# Autodesk Inventor assembly: Demonstrator
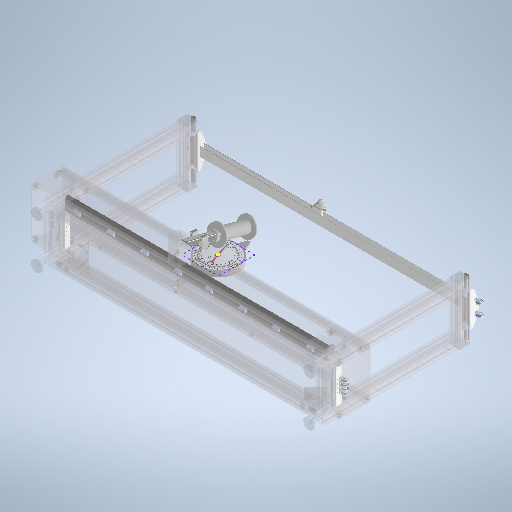
[picture p0: Inventor's stored thumbnail of the model, 512x512]
Saved by Autodesk Inventor 2025 (Build 290162010, 162A)
## iProperties
Created: 2024-11-07
Part Number: Demonstrator
Document SubType Name: Assembly
Designer: Admin
Mass: 7442.58 g
Surface Area: 46120.1 cm^2
Volume: 6360.4 cm^3
Density: 1.17015 g/cm^3
dummerWinkel: 1.5
Author: Admin
## Documents named in this file (38)
- C:\Users\Admin\GIT\HDVKBM\CAD\Krandemonstrator\Demonstrator.iam
- C:\Users\Admin\GIT\HDVKBM\CAD\Krandemonstrator\Träger.ipt
- C:\Users\Admin\Documents\Inventor\Content Center Files\R2025\de-DE\AS 1112 (2)\AS 1112 - M4  Typ 5.ipt
- C:\Users\Admin\GIT\HDVKBM\CAD\Krandemonstrator\MontageAufnahmeLO.ipt
- C:\Users\Admin\Documents\Inventor\Content Center Files\R2025\de-DE\AS 1427(03)\AS 1427 - M2 x 6(1).ipt
- C:\Users\Admin\GIT\HDVKBM\CAD\Krandemonstrator\Katze.iam
- C:\Users\Admin\GIT\HDVKBM\CAD\Krandemonstrator\UmlenkrolleHalterEinfach.iam
- C:\Users\Admin\GIT\HDVKBM\CAD\Krandemonstrator\SeilStange1m.ipt
- C:\Users\Admin\GIT\HDVKBM\CAD\Krandemonstrator\RollenhalterU.ipt
- C:\Users\Admin\GIT\HDVKBM\CAD\Krandemonstrator\UmlenkrolleHalterDoppelt.iam
- C:\Users\Admin\GIT\HDVKBM\CAD\Krandemonstrator\SeilatrappeHalter.ipt
- C:\Users\Admin\GIT\HDVKBM\CAD\Krandemonstrator\UmlenkrolleHalterDoppeltAngle.iam
- C:\Users\Admin\GIT\HDVKBM\CAD\Krandemonstrator\UmlenkrolleHalterEinfachAngle.iam
- C:\Users\Admin\GIT\HDVKBM\CAD\Krandemonstrator\UmlenkrolleHalterEinfachAngleB.iam
- C:\Users\Admin\GIT\HDVKBM\CAD\Krandemonstrator\seilatrappeHalterMini.ipt
- C:\Users\Admin\Documents\Inventor\Content Center Files\R2025\de-DE\AS 1421(4)\AS 1421 - M4 x 8 Kegelstumpf.ipt
- C:\Users\Admin\GIT\HDVKBM\CAD\Krandemonstrator\WS_10_40_930_2\WS_10_40_930_2.iam
- C:\Users\Admin\GIT\HDVKBM\CAD\Krandemonstrator\Frame.iam
- C:\Users\Admin\GIT\HDVKBM\CAD\Krandemonstrator\item_42006_nutenstein-8-st-m4-verzi__high\item_42006_nutenstein-8-st-m4-verzi__high.ipt
- C:\Users\Admin\Documents\Inventor\Content Center Files\R2025\de-DE\DIN 7991(2)\DIN 7991 - M4x30.ipt
- C:\Users\Admin\GIT\HDVKBM\CAD\Krandemonstrator\item_2623_nutenstein-8-st-m6-verzi__high\item_2623_nutenstein-8-st-m6-verzi__high.ipt
- C:\Users\Admin\Documents\Inventor\Content Center Files\R2025\de-DE\DIN 7991(2)\DIN 7991 - M6x16.ipt
- C:\Users\Admin\GIT\HDVKBM\CAD\Krandemonstrator\Zugfeder11.ipt
- C:\Users\Admin\GIT\HDVKBM\CAD\Krandemonstrator\Bedienhebel.iam
- C:\Users\Admin\Documents\Inventor\Content Center Files\R2025\de-DE\DIN 7991(1)\DIN 7991 - M4  x  25.ipt
- C:\Users\Admin\Documents\Inventor\Content Center Files\R2025\de-DE\DIN 7991(2)\DIN 7991 - M4x25.ipt
- C:\Users\Admin\GIT\HDVKBM\CAD\Krandemonstrator\SeilStange3cm.ipt
- C:\Users\Admin\GIT\HDVKBM\CAD\Krandemonstrator\waage.ipt
- C:\Users\Admin\GIT\HDVKBM\CAD\Krandemonstrator\verkleidungBremse.ipt
- C:\Users\Admin\Documents\Inventor\Content Center Files\R2025\de-DE\AS 1427(03)\AS 1427 - M2 x 4(1).ipt
- C:\Users\Admin\GIT\HDVKBM\CAD\Krandemonstrator\Platte Scharfe Ecken (mm) 150 x 30 x 8.ipt
- C:\Users\Admin\Documents\Inventor\Content Center Files\R2025\de-DE\DIN EN ISO 7089\DIN EN ISO 7089 -  5.ipt
- C:\Users\Admin\Documents\Inventor\Content Center Files\R2025\de-DE\DIN 933\DIN 933 - M5  x 8.ipt
- C:\Users\Admin\GIT\HDVKBM\CAD\Krandemonstrator\item_42005_nutenstein-8-st-m5-verzi__high\item_42005_nutenstein-8-st-m5-verzi__high.ipt
- C:\Users\Admin\Documents\Inventor\Content Center Files\R2025\de-DE\DIN 933\DIN 933 - M5  x 18.ipt
- C:\Users\Admin\GIT\HDVKBM\CAD\Krandemonstrator\MontageAufnahmeLO-LH.ipt
- C:\Users\Admin\Documents\Inventor\Content Center Files\R2025\de-DE\DIN 7991(1)\DIN 7991 - M3  x  16.ipt
- C:\Users\Admin\Documents\Inventor\Content Center Files\R2025\de-DE\DIN 7991(1)\DIN 7991 - M3  x  25.ipt
## Components (138 placed, 40 different names)
1. Katze:1 [sub-assembly] — KatzeLagerHO, KatzeLagerVV, KatzeSeilMutterVL, KatzeSeilMutterHL, KatzeSeilMutterVR, KatzeSeilMutterHR, KatzeGewindeSeilStumpfVL, KatzeGewindeSeilStumpfHL, KatzeGewindeSeilStumpfVR, KatzeGewindeSeilStumpfHR, KatzeSeilStumpfVL, KatzeSeilStumpfHL, KatzeSeilStumpfVR, KatzeSeilStumpfHR, Zylindrisch:83
2. Frame:1 [sub-assembly] — Starr:83, Starr:88, Starr:89, Starr:124, Starr:134, Starr:136
3. DIN EN ISO 7089 5:1
4. DIN EN ISO 7089 5:2
5. DIN EN ISO 7089 5:3
6. DIN EN ISO 7089 5:4
7. DIN 933 - ersetzt durch DIN EN 24017 M5  x 8:1
8. DIN 933 - ersetzt durch DIN EN 24017 M5  x 8:2 — Zylindrisch:109
9. DIN 933 - ersetzt durch DIN EN 24017 M5  x 8:3
10. DIN 933 - ersetzt durch DIN EN 24017 M5  x 8:4 — Zylindrisch:110
11. Platte Scharfe Ecken (mm) 150 x 30 x 8:2 — Starr:136, Einfügen:8, Zylindrisch:110
12. Platte Scharfe Ecken (mm) 150 x 30 x 8:1 — Starr:134, Zylindrisch:109, Planar:57
13. DIN 933 - ersetzt durch DIN EN 24017 M5  x 18:2
14. DIN 933 - ersetzt durch DIN EN 24017 M5  x 18:3
15. DIN 933 - ersetzt durch DIN EN 24017 M5  x 18:4
16. DIN 933 - ersetzt durch DIN EN 24017 M5  x 18:1 — Einfügen:8
17. DIN 7991 - ersetzt durch DIN EN ISO 10642 M3  x  16:4 — Passend:17
18. DIN 7991 - ersetzt durch DIN EN ISO 10642 M3  x  25:4 — Passend:18
19. DIN 7991 - ersetzt durch DIN EN ISO 10642 M3  x  25:3 — Passend:19
20. DIN 7991 - ersetzt durch DIN EN ISO 10642 M3  x  16:3 — Passend:20
21. DIN 7991 - ersetzt durch DIN EN ISO 10642 M3  x  16:2 — Passend:21
22. DIN 7991 - ersetzt durch DIN EN ISO 10642 M3  x  25:2 — Passend:22
23. DIN 7991 - ersetzt durch DIN EN ISO 10642 M3  x  16:1 — Passend:23
24. DIN 7991 - ersetzt durch DIN EN ISO 10642 M3  x  25:1 — Passend:24
25. MontageAufnahmeLO-LH:2 — SeilrolleORHscrewA, SeilrolleORHscrewB, SeilrolleORHplan, Starr:137, Passend:21, Passend:22
26. MontageAufnahmeLO:2 — SeilrolleORVplan, SeilrolleORVscrewA, SeilrolleORVscrewB, Starr:138, Passend:23, Passend:24
27. MontageAufnahmeLOV:1 — SeilrolleOLVAuflage, SeilrolleOLVSchraubeA, SeilrolleOLVSchraubeB, Starr:140, Passend:19, Passend:20
28. MontageAufnahmeLOH:1 — SeilrolleOLHAuflage, SeilrolleOLHSchraubeA, SeilrolleOLHSchraubeB, Starr:139, Passend:17, Passend:18
29. item_42005_nutenstein-8-st-m5-verzi__high:1
30. item_42005_nutenstein-8-st-m5-verzi__high:2
31. item_42005_nutenstein-8-st-m5-verzi__high:4
32. item_42005_nutenstein-8-st-m5-verzi__high:3
33. Träger:1 — KatzeLagerHO, KatzeLagerVV, Starr:137, Starr:138, Starr:139, Starr:140, Planar:57
34. Bedienhebel:1 [sub-assembly] — Passend:5, Passend:6, Passend:7, Passend:8, Kugelförmig:1, Kugelförmig:3
35. DIN 7991 - ersetzt durch DIN EN ISO 10642 M4  x  25:1 — Passend:5
36. DIN 7991 M4x25:1 — Passend:6
37. DIN 7991 M4x25:2 — Passend:7
38. DIN 7991 M4x25:3 — Passend:8
39. verkleidungBremse:1 — Passend:15, Passend:16
40. AS 1427 - Metrisch M2 x 4:1 — Passend:15
41. AS 1427 - Metrisch M2 x 4:2 — Passend:16
42. AS 1427 - Metrisch M2 x 4:3
43. AS 1427 - Metrisch M2 x 4:4
44. DIN 7991 M6x16:1 — Starr:90, Starr:105
45. DIN 7991 M6x16:2 — Starr:91, Starr:104
46. DIN 7991 M6x16:3 — Starr:93, Starr:102
47. DIN 7991 M6x16:4 — Starr:92, Starr:103
48. DIN 7991 M6x16:5 — Starr:97, Starr:98
49. DIN 7991 M6x16:6 — Starr:96, Starr:99
50. DIN 7991 M6x16:7 — Starr:95, Starr:100
51. DIN 7991 M6x16:8 — Starr:94, Starr:101
52. item_2623_nutenstein-8-st-m6-verzi__high:1 — Starr:105
53. item_2623_nutenstein-8-st-m6-verzi__high:2 — Starr:104
54. item_2623_nutenstein-8-st-m6-verzi__high:3 — Starr:99
55. item_2623_nutenstein-8-st-m6-verzi__high:4 — Starr:103
56. item_2623_nutenstein-8-st-m6-verzi__high:5 — Starr:102
57. item_2623_nutenstein-8-st-m6-verzi__high:6 — Starr:101
58. item_2623_nutenstein-8-st-m6-verzi__high:7 — Starr:100
59. item_2623_nutenstein-8-st-m6-verzi__high:8 — Starr:98
60. WS_10_40_930_2:1 [sub-assembly] — Starr:89, Starr:90, Starr:91, Starr:92, Starr:93, Starr:94, Starr:95, Starr:96, Starr:97
61. lastseil — Zylindrisch:83, Starr:117
62. Zugfeder1:1 — Starr:118
63. waage:1 — Starr:117, Starr:118
64. SeilStange3cm:5 — Starr:119, Kugelförmig:3
65. SeilStange3cm:6 — Starr:119
66. SeilStange3cm:7 — Starr:122
67. SeilStange3cm:8 — Starr:122, Starr:123
68. SeilStange3cm:2 — Zylindrisch:108
69. SeilStange3cm:1 — Kugelförmig:1, Zylindrisch:108, Starr:123
70. seilatrappeHalterMini:3 — SeilAtrappeHalterMini3, SeilAtrappeHalterMini3Seil
71. seilatrappeHalterMini:4 — SeilAtrappeHalterMini4, SeilAtrappeHalterMini4Seil
72. SeilStange1m:16 — SeilrolleULMVsld, SeilAtrappeHalterMini3Seil
73. SeilStange1m:17 — SeilrolleULMHsld, SeilAtrappeHalterMini4Seil
74. SeilStange1m:18 — SeilAtrappeHalterMini1Seil, SeilrolleORVver, SeilrolleURMVver
75. SeilStange1m:19 — SeilAtrappeHalterMini2Seil, SeilrolleORHver, SeilrolleURMHver
76. seilatrappeHalterMini:1 — SeilAtrappeHalterMini1, SeilAtrappeHalterMini1Seil
77. seilatrappeHalterMini:2 — SeilAtrappeHalterMini2, SeilAtrappeHalterMini2Seil
78. SeilStange1m:13 — SeilrolleURHsld
79. SeilStange1m:12 — SeilrolleURVsld
80. SeilatrappeHalter:1 — SeilAtrappeHalterSeilA, SeilAtrappeHalterSeilB, Starr:124
81. SeilStange1m:1 — KatzeGewindeSeilStumpfVL, SeilrolleOLVhor
82. SeilStange1m:3 — SeilrolleOLHhor, KatzeSeilStumpfHL
83. SeilStange1m:4 — SeilrolleORHhor, KatzeSeilStumpfHR
84. SeilStange1m:5 — SeilrolleORVhor, KatzeSeilStumpfVR
85. SeilStange1m:8 — SeilAtrappeHalterSeilB, SeilrolleOLHver, SeilrolleULHver
86. SeilStange1m:9 — SeilAtrappeHalterSeilA, SeilrolleOLVver, SeilrolleULVver
87. SeilStange1m:10 — Zylindrisch:15, SeilrolleULHhor, SeilrolleURHhor
88. SeilStange1m:11 — Zylindrisch:16, SeilrolleULVhor, SeilrolleURVhor
89. SeilStange1m:14 — SeilAtrappeRollenhalterSeilB, SeilrolleULMHhor, SeilrolleURMHhor
90. SeilStange1m:15 — SeilAtrappeRollenhalterSeilA, SeilrolleULMVhor, SeilrolleURMVhor
91. AS 1427 - Metrisch M2 x 6:2 — SeilrolleOLVSchraube2, SeilrolleOLVSchraubeA
92. AS 1427 - Metrisch M2 x 6:1 — SeilrolleOLVSchraube1, SeilrolleOLVSchraubeB
93. UmlenkrolleHalterEinfach:1 [sub-assembly] — SeilrolleOLVSchraube1, SeilrolleOLVAuflage, SeilrolleOLVSchraube2, SeilrolleOLVhor, SeilrolleOLVver
94. AS 1427 - Metrisch M2 x 6:3 — SeilrolleOLHSchraube1, SeilrolleOLHSchraubeA
95. AS 1427 - Metrisch M2 x 6:4 — SeilrolleOLHSchraube2, SeilrolleOLHSchraubeB
96. UmlenkrolleHalterEinfach:2 [sub-assembly] — SeilrolleOLHSchraube1, SeilrolleOLHSchraube2, SeilrolleOLHAuflage, SeilrolleOLHhor, SeilrolleOLHver
97. AS 1112 (2) - Metrisch M4  Typ 5:4 — KatzeSeilMutterVR
98. AS 1112 (2) - Metrisch M4  Typ 5:3 — KatzeSeilMutterVL
99. AS 1112 (2) - Metrisch M4  Typ 5:2 — KatzeSeilMutterHR
100. AS 1112 (2) - Metrisch M4  Typ 5:1 — KatzeSeilMutterHL
101. AS 1421 Kegelstumpf - Metrisch M4 x 8 Kegelstumpf:4 — KatzeGewindeSeilStumpfHR
102. AS 1421 Kegelstumpf - Metrisch M4 x 8 Kegelstumpf:1 — KatzeGewindeSeilStumpfVR
103. AS 1421 Kegelstumpf - Metrisch M4 x 8 Kegelstumpf:2 — KatzeSeilStumpfVL
104. AS 1421 Kegelstumpf - Metrisch M4 x 8 Kegelstumpf:3 — KatzeGewindeSeilStumpfHL
105. UmlenkrolleHalterEinfachAngle:1 [sub-assembly] — SeilrolleORVscrewAfix, SeilrolleORVscrewBfix, SeilrolleORVplan, SeilrolleORVhor, SeilrolleORVver, SeilAtrappeHalterMini1
106. AS 1427 - Metrisch M2 x 6:17 — SeilrolleORVscrewBfix, SeilrolleORVscrewB
107. AS 1427 - Metrisch M2 x 6:18 — SeilrolleORVscrewAfix, SeilrolleORVscrewA
108. AS 1427 - Metrisch M2 x 6:19 — SeilrolleORHscrewB, SeilrolleORHscrewBfix
109. AS 1427 - Metrisch M2 x 6:20 — SeilrolleORHscrewA, SeilrolleORHscrewAfix
110. UmlenkrolleHalterEinfachAngleB:1 [sub-assembly] — SeilrolleORHplan, SeilrolleORHscrewAfix, SeilrolleORHscrewBfix, SeilAtrappeHalterMini2, SeilrolleORHhor, SeilrolleORHver
111. RollenhalterU:1 — Planar:24, Zylindrisch:5, Zylindrisch:6, Planar:25, Zylindrisch:7, Zylindrisch:8, Planar:40, Zylindrisch:9, Zylindrisch:10, Zylindrisch:15, Zylindrisch:16, Starr:84, Starr:85, Passend:1, Passend:2, Starr:88
112. DIN 7991 M4x30:1 — Passend:1
113. DIN 7991 M4x30:2 — Passend:2
114. UmlenkrolleHalterDoppelt:1 [sub-assembly] — Planar:24, Starr:33, Starr:34, SeilrolleULMHhor, SeilrolleULMVhor, SeilrolleULMHsld, SeilrolleULMVsld, SeilAtrappeHalterMini3, SeilAtrappeHalterMini4
115. UmlenkrolleHalterEinfach:3 [sub-assembly] — Starr:35, Starr:36, Planar:25, SeilrolleULVver, SeilrolleULVhor
116. UmlenkrolleHalterEinfach:4 [sub-assembly] — Starr:37, Starr:38, Planar:40, SeilrolleULHver, SeilrolleULHhor
117. AS 1427 - Metrisch M2 x 6:5 — Starr:38, Zylindrisch:9
118. AS 1427 - Metrisch M2 x 6:6 — Starr:37, Zylindrisch:10
119. AS 1427 - Metrisch M2 x 6:7 — Starr:34, Zylindrisch:6
120. AS 1427 - Metrisch M2 x 6:8 — Starr:33, Zylindrisch:5
121. AS 1427 - Metrisch M2 x 6:9 — Starr:35, Zylindrisch:8
122. item_42006_nutenstein-8-st-m4-verzi__high:1 — Starr:85
123. item_42006_nutenstein-8-st-m4-verzi__high:2 — Starr:84
124. AS 1427 - Metrisch M2 x 6:10 — Starr:36, Zylindrisch:7
125. UmlenkrolleHalterEinfach:5 [sub-assembly] — Starr:45, Starr:44, Planar:42, SeilrolleURVhor, SeilrolleURVsld
126. UmlenkrolleHalterEinfach:6 [sub-assembly] — Starr:46, Starr:47, Planar:43, SeilrolleURHhor, SeilrolleURHsld
127. UmlenkrolleHalterDoppeltAngle:1 [sub-assembly] — Planar:54, Starr:53, Starr:54, SeilrolleURMHhor, SeilrolleURMVhor, SeilrolleURMVver, SeilrolleURMHver
128. AS 1427 - Metrisch M2 x 6:11 — Starr:47, Zylindrisch:22
129. AS 1427 - Metrisch M2 x 6:12 — Starr:46, Zylindrisch:21
130. AS 1427 - Metrisch M2 x 6:13 — Starr:45, Zylindrisch:20
131. AS 1427 - Metrisch M2 x 6:14 — Zylindrisch:18, Starr:53
132. AS 1427 - Metrisch M2 x 6:15 — Zylindrisch:17, Starr:54
133. AS 1427 - Metrisch M2 x 6:16 — Starr:44, Zylindrisch:19
134. RollenhalterU:2 — Zylindrisch:17, Zylindrisch:18, Planar:42, Zylindrisch:19, Zylindrisch:20, Planar:43, Zylindrisch:21, Zylindrisch:22, Planar:54, SeilAtrappeRollenhalterSeilB, SeilAtrappeRollenhalterSeilA, Starr:83, Passend:3, Passend:4, Starr:86, Starr:87
135. DIN 7991 M4x30:3 — Passend:3
136. item_42006_nutenstein-8-st-m4-verzi__high:3 — Starr:87
137. item_42006_nutenstein-8-st-m4-verzi__high:4 — Starr:86
138. DIN 7991 M4x30:4 — Passend:4
## Relationships (174: WeldJoint 75, CylindricalJoint 34, RelateRotateTranslate 24, Mate 18, PlanarJoint 13, Insert 8, BallJoint 2)
- KatzeLagerHO [PlanarJoint] (0.05 mm): Katze:1 ↔ Träger:1
- KatzeLagerVV [PlanarJoint] (0.05 mm): Katze:1 ↔ Träger:1
- KatzeSeilMutterVL [WeldJoint]: Katze:1 ↔ AS 1112 (2) - Metrisch M4  Typ 5:3
- KatzeSeilMutterHL [WeldJoint]: Katze:1 ↔ AS 1112 (2) - Metrisch M4  Typ 5:1
- KatzeSeilMutterVR [WeldJoint]: Katze:1 ↔ AS 1112 (2) - Metrisch M4  Typ 5:4
- KatzeSeilMutterHR [WeldJoint]: Katze:1 ↔ AS 1112 (2) - Metrisch M4  Typ 5:2
- KatzeGewindeSeilStumpfVL [WeldJoint]: Katze:1 ↔ SeilStange1m:1
- KatzeGewindeSeilStumpfHL [WeldJoint]: Katze:1 ↔ AS 1421 Kegelstumpf - Metrisch M4 x 8 Kegelstumpf:3
- KatzeGewindeSeilStumpfVR [WeldJoint]: Katze:1 ↔ AS 1421 Kegelstumpf - Metrisch M4 x 8 Kegelstumpf:1
- KatzeGewindeSeilStumpfHR [WeldJoint]: Katze:1 ↔ AS 1421 Kegelstumpf - Metrisch M4 x 8 Kegelstumpf:4
- KatzeSeilStumpfVL [WeldJoint]: Katze:1 ↔ AS 1421 Kegelstumpf - Metrisch M4 x 8 Kegelstumpf:2
- KatzeSeilStumpfHL [WeldJoint]: Katze:1 ↔ SeilStange1m:3
- KatzeSeilStumpfVR [WeldJoint]: Katze:1 ↔ SeilStange1m:5
- KatzeSeilStumpfHR [WeldJoint]: Katze:1 ↔ SeilStange1m:4
- SeilrolleOLVSchraube1 [WeldJoint]: AS 1427 - Metrisch M2 x 6:1 ↔ UmlenkrolleHalterEinfach:1
- SeilrolleOLVSchraube2 [WeldJoint]: AS 1427 - Metrisch M2 x 6:2 ↔ UmlenkrolleHalterEinfach:1
- SeilrolleOLVAuflage [PlanarJoint]: MontageAufnahmeLOV:1 ↔ UmlenkrolleHalterEinfach:1
- SeilrolleOLVSchraubeA [CylindricalJoint]: MontageAufnahmeLOV:1 ↔ AS 1427 - Metrisch M2 x 6:2
- SeilrolleOLVSchraubeB [CylindricalJoint]: MontageAufnahmeLOV:1 ↔ AS 1427 - Metrisch M2 x 6:1
- SeilrolleOLVhor [RelateRotateTranslate] (9 mm): SeilStange1m:1 ↔ UmlenkrolleHalterEinfach:1
- SeilrolleOLVver [RelateRotateTranslate] (9 mm): SeilStange1m:9 ↔ UmlenkrolleHalterEinfach:1
- SeilrolleOLHSchraube1 [WeldJoint]: AS 1427 - Metrisch M2 x 6:3 ↔ UmlenkrolleHalterEinfach:2
- SeilrolleOLHSchraube2 [WeldJoint]: AS 1427 - Metrisch M2 x 6:4 ↔ UmlenkrolleHalterEinfach:2
- SeilrolleOLHAuflage [PlanarJoint]: MontageAufnahmeLOH:1 ↔ UmlenkrolleHalterEinfach:2
- SeilrolleOLHSchraubeA [CylindricalJoint]: MontageAufnahmeLOH:1 ↔ AS 1427 - Metrisch M2 x 6:3
- SeilrolleOLHSchraubeB [CylindricalJoint]: MontageAufnahmeLOH:1 ↔ AS 1427 - Metrisch M2 x 6:4
- SeilrolleOLHhor [RelateRotateTranslate] (9 mm): SeilStange1m:3 ↔ UmlenkrolleHalterEinfach:2
- SeilrolleOLHver [RelateRotateTranslate] (9 mm): SeilStange1m:8 ↔ UmlenkrolleHalterEinfach:2
- Planar:24: RollenhalterU:1 ↔ UmlenkrolleHalterDoppelt:1
- Starr:33 [WeldJoint]: UmlenkrolleHalterDoppelt:1 ↔ AS 1427 - Metrisch M2 x 6:8
- Starr:34 [WeldJoint]: UmlenkrolleHalterDoppelt:1 ↔ AS 1427 - Metrisch M2 x 6:7
- Zylindrisch:5 [CylindricalJoint]: RollenhalterU:1 ↔ AS 1427 - Metrisch M2 x 6:8
- Zylindrisch:6 [CylindricalJoint]: RollenhalterU:1 ↔ AS 1427 - Metrisch M2 x 6:7
- Starr:35 [WeldJoint]: UmlenkrolleHalterEinfach:3 ↔ AS 1427 - Metrisch M2 x 6:9
- Starr:36 [WeldJoint]: UmlenkrolleHalterEinfach:3 ↔ AS 1427 - Metrisch M2 x 6:10
- Planar:25: RollenhalterU:1 ↔ UmlenkrolleHalterEinfach:3
- Zylindrisch:7 [CylindricalJoint]: RollenhalterU:1 ↔ AS 1427 - Metrisch M2 x 6:10
- Zylindrisch:8 [CylindricalJoint]: RollenhalterU:1 ↔ AS 1427 - Metrisch M2 x 6:9
- Starr:37 [WeldJoint]: UmlenkrolleHalterEinfach:4 ↔ AS 1427 - Metrisch M2 x 6:6
- Starr:38 [WeldJoint]: UmlenkrolleHalterEinfach:4 ↔ AS 1427 - Metrisch M2 x 6:5
- Planar:40: RollenhalterU:1 ↔ UmlenkrolleHalterEinfach:4
- Zylindrisch:9 [CylindricalJoint]: RollenhalterU:1 ↔ AS 1427 - Metrisch M2 x 6:5
- Zylindrisch:10 [CylindricalJoint]: RollenhalterU:1 ↔ AS 1427 - Metrisch M2 x 6:6
- SeilAtrappeHalterSeilA [CylindricalJoint]: SeilatrappeHalter:1 ↔ SeilStange1m:9
- SeilAtrappeHalterSeilB [CylindricalJoint]: SeilatrappeHalter:1 ↔ SeilStange1m:8
- Zylindrisch:15 [CylindricalJoint]: SeilStange1m:10 ↔ RollenhalterU:1
- Zylindrisch:16 [CylindricalJoint]: SeilStange1m:11 ↔ RollenhalterU:1
- SeilrolleULVver [RelateRotateTranslate] (9 mm): SeilStange1m:9 ↔ UmlenkrolleHalterEinfach:3
- SeilrolleULHver [RelateRotateTranslate] (9 mm): SeilStange1m:8 ↔ UmlenkrolleHalterEinfach:4
- SeilrolleULVhor [RelateRotateTranslate] (9 mm): SeilStange1m:11 ↔ UmlenkrolleHalterEinfach:3
- SeilrolleULHhor [RelateRotateTranslate] (9 mm): SeilStange1m:10 ↔ UmlenkrolleHalterEinfach:4
- Zylindrisch:17 [CylindricalJoint]: AS 1427 - Metrisch M2 x 6:15 ↔ RollenhalterU:2
- Zylindrisch:18 [CylindricalJoint]: AS 1427 - Metrisch M2 x 6:14 ↔ RollenhalterU:2
- Starr:45 [WeldJoint]: UmlenkrolleHalterEinfach:5 ↔ AS 1427 - Metrisch M2 x 6:13
- Starr:44 [WeldJoint]: UmlenkrolleHalterEinfach:5 ↔ AS 1427 - Metrisch M2 x 6:16
- Planar:42: UmlenkrolleHalterEinfach:5 ↔ RollenhalterU:2
- Zylindrisch:19 [CylindricalJoint]: AS 1427 - Metrisch M2 x 6:16 ↔ RollenhalterU:2
- Zylindrisch:20 [CylindricalJoint]: AS 1427 - Metrisch M2 x 6:13 ↔ RollenhalterU:2
- Starr:46 [WeldJoint]: UmlenkrolleHalterEinfach:6 ↔ AS 1427 - Metrisch M2 x 6:12
- Starr:47 [WeldJoint]: UmlenkrolleHalterEinfach:6 ↔ AS 1427 - Metrisch M2 x 6:11
- Planar:43: UmlenkrolleHalterEinfach:6 ↔ RollenhalterU:2
- Zylindrisch:21 [CylindricalJoint]: AS 1427 - Metrisch M2 x 6:12 ↔ RollenhalterU:2
- Zylindrisch:22 [CylindricalJoint]: AS 1427 - Metrisch M2 x 6:11 ↔ RollenhalterU:2
- SeilrolleURHhor [RelateRotateTranslate] (9 mm): SeilStange1m:10 ↔ UmlenkrolleHalterEinfach:6
- SeilrolleURVhor [RelateRotateTranslate] (9 mm): SeilStange1m:11 ↔ UmlenkrolleHalterEinfach:5
- SeilrolleURVsld [RelateRotateTranslate] (9 mm): SeilStange1m:12 ↔ UmlenkrolleHalterEinfach:5
- SeilrolleURHsld [RelateRotateTranslate] (9 mm): SeilStange1m:13 ↔ UmlenkrolleHalterEinfach:6
- Planar:54: UmlenkrolleHalterDoppeltAngle:1 ↔ RollenhalterU:2
- Starr:53 [WeldJoint]: UmlenkrolleHalterDoppeltAngle:1 ↔ AS 1427 - Metrisch M2 x 6:14
- Starr:54 [WeldJoint]: UmlenkrolleHalterDoppeltAngle:1 ↔ AS 1427 - Metrisch M2 x 6:15
- SeilrolleORVscrewAfix [WeldJoint]: UmlenkrolleHalterEinfachAngle:1 ↔ AS 1427 - Metrisch M2 x 6:18
- SeilrolleORVscrewBfix [WeldJoint]: UmlenkrolleHalterEinfachAngle:1 ↔ AS 1427 - Metrisch M2 x 6:17
- SeilrolleORVplan [PlanarJoint]: MontageAufnahmeLO:2 ↔ UmlenkrolleHalterEinfachAngle:1
- SeilrolleORVscrewA [CylindricalJoint]: MontageAufnahmeLO:2 ↔ AS 1427 - Metrisch M2 x 6:18
- SeilrolleORVscrewB [CylindricalJoint]: MontageAufnahmeLO:2 ↔ AS 1427 - Metrisch M2 x 6:17
- SeilrolleORHscrewA [CylindricalJoint]: MontageAufnahmeLO-LH:2 ↔ AS 1427 - Metrisch M2 x 6:20
- SeilrolleORHscrewB [CylindricalJoint]: MontageAufnahmeLO-LH:2 ↔ AS 1427 - Metrisch M2 x 6:19
- SeilrolleORHplan [PlanarJoint]: MontageAufnahmeLO-LH:2 ↔ UmlenkrolleHalterEinfachAngleB:1
- SeilrolleORHscrewAfix [WeldJoint]: AS 1427 - Metrisch M2 x 6:20 ↔ UmlenkrolleHalterEinfachAngleB:1
- SeilrolleORHscrewBfix [WeldJoint]: AS 1427 - Metrisch M2 x 6:19 ↔ UmlenkrolleHalterEinfachAngleB:1
- SeilAtrappeRollenhalterSeilB [CylindricalJoint]: SeilStange1m:14 ↔ RollenhalterU:2
- SeilAtrappeRollenhalterSeilA [CylindricalJoint]: SeilStange1m:15 ↔ RollenhalterU:2
- SeilrolleORHhor [RelateRotateTranslate] (9 mm): SeilStange1m:4 ↔ UmlenkrolleHalterEinfachAngleB:1
- SeilrolleORVhor [RelateRotateTranslate] (9 mm): SeilStange1m:5 ↔ UmlenkrolleHalterEinfachAngle:1
- SeilrolleORHver [RelateRotateTranslate] (9 mm): SeilStange1m:19 ↔ UmlenkrolleHalterEinfachAngleB:1
- SeilrolleORVver [RelateRotateTranslate] (9 mm): SeilStange1m:18 ↔ UmlenkrolleHalterEinfachAngle:1
- SeilrolleURMHhor [RelateRotateTranslate] (9 mm): SeilStange1m:14 ↔ UmlenkrolleHalterDoppeltAngle:1
- SeilrolleURMVhor [RelateRotateTranslate] (9 mm): SeilStange1m:15 ↔ UmlenkrolleHalterDoppeltAngle:1
- SeilrolleURMVver [RelateRotateTranslate] (9 mm): SeilStange1m:18 ↔ UmlenkrolleHalterDoppeltAngle:1
- SeilrolleURMHver [RelateRotateTranslate] (9 mm): SeilStange1m:19 ↔ UmlenkrolleHalterDoppeltAngle:1
- SeilrolleULMHhor [RelateRotateTranslate] (9 mm): SeilStange1m:14 ↔ UmlenkrolleHalterDoppelt:1
- SeilrolleULMVhor [RelateRotateTranslate] (9 mm): SeilStange1m:15 ↔ UmlenkrolleHalterDoppelt:1
- SeilrolleULMHsld [RelateRotateTranslate] (9 mm): SeilStange1m:17 ↔ UmlenkrolleHalterDoppelt:1
- SeilrolleULMVsld [RelateRotateTranslate] (9 mm): SeilStange1m:16 ↔ UmlenkrolleHalterDoppelt:1
- SeilAtrappeHalterMini1 [WeldJoint]: seilatrappeHalterMini:1 ↔ UmlenkrolleHalterEinfachAngle:1
- SeilAtrappeHalterMini1Seil [CylindricalJoint]: SeilStange1m:18 ↔ seilatrappeHalterMini:1
- SeilAtrappeHalterMini2 [WeldJoint]: seilatrappeHalterMini:2 ↔ UmlenkrolleHalterEinfachAngleB:1
- SeilAtrappeHalterMini2Seil [CylindricalJoint]: SeilStange1m:19 ↔ seilatrappeHalterMini:2
- SeilAtrappeHalterMini3 [WeldJoint]: seilatrappeHalterMini:3 ↔ UmlenkrolleHalterDoppelt:1
- SeilAtrappeHalterMini3Seil [CylindricalJoint]: seilatrappeHalterMini:3 ↔ SeilStange1m:16
- SeilAtrappeHalterMini4 [WeldJoint]: seilatrappeHalterMini:4 ↔ UmlenkrolleHalterDoppelt:1
- SeilAtrappeHalterMini4Seil [CylindricalJoint]: seilatrappeHalterMini:4 ↔ SeilStange1m:17
- Zylindrisch:83 [CylindricalJoint]: Katze:1 ↔ lastseil
- Starr:83 [WeldJoint]: Frame:1 ↔ RollenhalterU:2
- Starr:84 [WeldJoint]: RollenhalterU:1 ↔ item_42006_nutenstein-8-st-m4-verzi__high:2
- Starr:85 [WeldJoint]: RollenhalterU:1 ↔ item_42006_nutenstein-8-st-m4-verzi__high:1
- Passend:1 [Mate]: RollenhalterU:1 ↔ DIN 7991 M4x30:1
- Passend:2 [Mate]: RollenhalterU:1 ↔ DIN 7991 M4x30:2
- Passend:3 [Mate]: RollenhalterU:2 ↔ DIN 7991 M4x30:3
- Passend:4 [Mate]: RollenhalterU:2 ↔ DIN 7991 M4x30:4
- Starr:86 [WeldJoint]: RollenhalterU:2 ↔ item_42006_nutenstein-8-st-m4-verzi__high:4
- Starr:87 [WeldJoint]: RollenhalterU:2 ↔ item_42006_nutenstein-8-st-m4-verzi__high:3
- Starr:88 [WeldJoint]: Frame:1 ↔ RollenhalterU:1
- Starr:89 [WeldJoint] (1.5 mm): Frame:1 ↔ WS_10_40_930_2:1
- Starr:90 [WeldJoint]: DIN 7991 M6x16:1 ↔ WS_10_40_930_2:1
- Starr:91 [WeldJoint]: DIN 7991 M6x16:2 ↔ WS_10_40_930_2:1
- Starr:92 [WeldJoint]: DIN 7991 M6x16:4 ↔ WS_10_40_930_2:1
- Starr:93 [WeldJoint]: DIN 7991 M6x16:3 ↔ WS_10_40_930_2:1
- Starr:94 [WeldJoint]: DIN 7991 M6x16:8 ↔ WS_10_40_930_2:1
- Starr:95 [WeldJoint]: DIN 7991 M6x16:7 ↔ WS_10_40_930_2:1
- Starr:96 [WeldJoint]: DIN 7991 M6x16:6 ↔ WS_10_40_930_2:1
- Starr:97 [WeldJoint]: DIN 7991 M6x16:5 ↔ WS_10_40_930_2:1
- Starr:98 [WeldJoint]: DIN 7991 M6x16:5 ↔ item_2623_nutenstein-8-st-m6-verzi__high:8
- Starr:99 [WeldJoint]: DIN 7991 M6x16:6 ↔ item_2623_nutenstein-8-st-m6-verzi__high:3
- Starr:100 [WeldJoint]: DIN 7991 M6x16:7 ↔ item_2623_nutenstein-8-st-m6-verzi__high:7
- Starr:101 [WeldJoint]: DIN 7991 M6x16:8 ↔ item_2623_nutenstein-8-st-m6-verzi__high:6
- Starr:102 [WeldJoint]: DIN 7991 M6x16:3 ↔ item_2623_nutenstein-8-st-m6-verzi__high:5
- Starr:103 [WeldJoint]: DIN 7991 M6x16:4 ↔ item_2623_nutenstein-8-st-m6-verzi__high:4
- Starr:104 [WeldJoint]: DIN 7991 M6x16:2 ↔ item_2623_nutenstein-8-st-m6-verzi__high:2
- Starr:105 [WeldJoint]: DIN 7991 M6x16:1 ↔ item_2623_nutenstein-8-st-m6-verzi__high:1
- Passend:5 [Mate]: Bedienhebel:1 ↔ DIN 7991 - ersetzt durch DIN EN ISO 10642 M4  x  25:1
- Passend:6 [Mate]: Bedienhebel:1 ↔ DIN 7991 M4x25:1
- Passend:7 [Mate]: Bedienhebel:1 ↔ DIN 7991 M4x25:2
- Passend:8 [Mate]: Bedienhebel:1 ↔ DIN 7991 M4x25:3
- Zylindrisch:108 [CylindricalJoint]: SeilStange3cm:2 ↔ SeilStange3cm:1
- Kugelförmig:1 [BallJoint]: Bedienhebel:1 ↔ SeilStange3cm:1
- Starr:117 [WeldJoint] (-430 mm): lastseil ↔ waage:1
- Starr:118 [WeldJoint]: Zugfeder1:1 ↔ waage:1
- Starr:119 [WeldJoint] (6.3883 mm): SeilStange3cm:5 ↔ SeilStange3cm:6
- Kugelförmig:3 [BallJoint]: Bedienhebel:1 ↔ SeilStange3cm:5
- Starr:122 [WeldJoint]: SeilStange3cm:7 ↔ SeilStange3cm:8
- Starr:123 [WeldJoint]: SeilStange3cm:8 ↔ SeilStange3cm:1
- Starr:124 [WeldJoint]: Frame:1 ↔ SeilatrappeHalter:1
- Passend:15 [Mate]: verkleidungBremse:1 ↔ AS 1427 - Metrisch M2 x 4:1
- Passend:16 [Mate]: verkleidungBremse:1 ↔ AS 1427 - Metrisch M2 x 4:2
- [WeldJoint]: DIN EN ISO 7089 5:1 ↔ Träger:1
- [WeldJoint]: DIN EN ISO 7089 5:2 ↔ Träger:1
- [WeldJoint]: DIN EN ISO 7089 5:4 ↔ Träger:1
- [WeldJoint]: DIN EN ISO 7089 5:3 ↔ Träger:1
- Starr:134 [WeldJoint]: Frame:1 ↔ Platte Scharfe Ecken (mm) 150 x 30 x 8:1
- [Insert]: DIN EN ISO 7089 5:3 ↔ DIN 933 - ersetzt durch DIN EN 24017 M5  x 8:1
- [Insert]: DIN EN ISO 7089 5:4 ↔ DIN 933 - ersetzt durch DIN EN 24017 M5  x 8:2
- [Insert]: DIN EN ISO 7089 5:2 ↔ DIN 933 - ersetzt durch DIN EN 24017 M5  x 8:3
- [Insert]: DIN EN ISO 7089 5:1 ↔ DIN 933 - ersetzt durch DIN EN 24017 M5  x 8:4
- Starr:136 [WeldJoint]: Frame:1 ↔ Platte Scharfe Ecken (mm) 150 x 30 x 8:2
- [Insert]: Platte Scharfe Ecken (mm) 150 x 30 x 8:1 ↔ DIN 933 - ersetzt durch DIN EN 24017 M5  x 18:2
- [Insert]: Platte Scharfe Ecken (mm) 150 x 30 x 8:1 ↔ DIN 933 - ersetzt durch DIN EN 24017 M5  x 18:3
- [Insert]: Platte Scharfe Ecken (mm) 150 x 30 x 8:2 ↔ DIN 933 - ersetzt durch DIN EN 24017 M5  x 18:4
- Einfügen:8 [Insert]: Platte Scharfe Ecken (mm) 150 x 30 x 8:2 ↔ DIN 933 - ersetzt durch DIN EN 24017 M5  x 18:1
- Starr:137 [WeldJoint]: MontageAufnahmeLO-LH:2 ↔ Träger:1
- Starr:138 [WeldJoint]: MontageAufnahmeLO:2 ↔ Träger:1
- Starr:139 [WeldJoint]: MontageAufnahmeLOH:1 ↔ Träger:1
- Starr:140 [WeldJoint]: MontageAufnahmeLOV:1 ↔ Träger:1
- Passend:17 [Mate]: DIN 7991 - ersetzt durch DIN EN ISO 10642 M3  x  16:4 ↔ MontageAufnahmeLOH:1
- Passend:18 [Mate]: DIN 7991 - ersetzt durch DIN EN ISO 10642 M3  x  25:4 ↔ MontageAufnahmeLOH:1
- Passend:19 [Mate]: DIN 7991 - ersetzt durch DIN EN ISO 10642 M3  x  25:3 ↔ MontageAufnahmeLOV:1
- Passend:20 [Mate]: DIN 7991 - ersetzt durch DIN EN ISO 10642 M3  x  16:3 ↔ MontageAufnahmeLOV:1
- Passend:21 [Mate]: DIN 7991 - ersetzt durch DIN EN ISO 10642 M3  x  16:2 ↔ MontageAufnahmeLO-LH:2
- Passend:22 [Mate]: DIN 7991 - ersetzt durch DIN EN ISO 10642 M3  x  25:2 ↔ MontageAufnahmeLO-LH:2
- Passend:23 [Mate]: DIN 7991 - ersetzt durch DIN EN ISO 10642 M3  x  16:1 ↔ MontageAufnahmeLO:2
- Passend:24 [Mate]: DIN 7991 - ersetzt durch DIN EN ISO 10642 M3  x  25:1 ↔ MontageAufnahmeLO:2
- Zylindrisch:109 [CylindricalJoint]: DIN 933 - ersetzt durch DIN EN 24017 M5  x 8:2 ↔ Platte Scharfe Ecken (mm) 150 x 30 x 8:1
- Planar:57: Platte Scharfe Ecken (mm) 150 x 30 x 8:1 ↔ Träger:1
- Zylindrisch:110 [CylindricalJoint]: DIN 933 - ersetzt durch DIN EN 24017 M5  x 8:4 ↔ Platte Scharfe Ecken (mm) 150 x 30 x 8:2
## Named parameters: Finish2_Area = 2136.28, Finish3_Area = 43.5425, Finish4_Area = 0.0628319
note: some values were not read from the file. Shown as the stored number, unit unknown: "Finish2_Area", "Finish3_Area", "Finish4_Area".
